# Autodesk Inventor assembly: Side Lidar Assembly
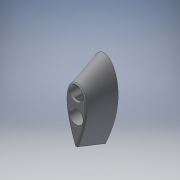
[picture p0: Inventor's stored thumbnail of the model, 180x180]
Saved by Autodesk Inventor 2016 (Build 200138000, 138)
## iProperties
Created: 2017-05-14
Part Number: Side Lidar Assembly
Document SubType Name: Assembly
Designer: BenjaPad
Author: BenjaPad
## Documents named in this file (5)
- C:\Users\BenjaPad\Google Drev\Bachelor\Teststand\Elektro 3D print\Side Lidar Assembly.iam
- C:\Users\BenjaPad\Google Drev\Bachelor\Teststand\Elektro 3D print\Aero Lidar Mount.ipt
- C:\Users\BenjaPad\Google Drev\Bachelor\Teststand\Elektro 3D print\Side Lidar.ipt
- C:\Users\BenjaPad\Google Drev\Bachelor\Teststand\Elektro 3D print\Aero Lidar Pod.ipt
- C:\Users\BenjaPad\Google Drev\Bachelor\Teststand\Elektro 3D print\Aero Lidar bracket mount.ipt
## Components (4 placed, 4 different names)
1. Aero Lidar Mount:1 — Flush:1, Flush:2, Flush:3, Flush:4
2. Side Lidar:1 — Flush:4, Flush:5
3. Aero Lidar Pod:1 — Flush:5, Flush:6
4. Aero Lidar bracket mount:1 — Flush:6
## Relationships (6: Flush 6)
- Flush:1: Aero Lidar Mount:1
- Flush:2: Aero Lidar Mount:1
- Flush:3: Aero Lidar Mount:1
- Flush:4: Aero Lidar Mount:1 ↔ Side Lidar:1
- Flush:5: Side Lidar:1 ↔ Aero Lidar Pod:1
- Flush:6: Aero Lidar Pod:1 ↔ Aero Lidar bracket mount:1
